# Autodesk Inventor assembly: Extrusions (1)
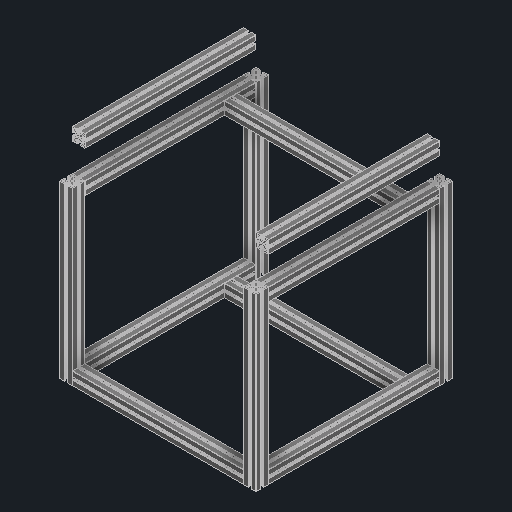
[picture p0: Inventor's stored thumbnail of the model, 512x512]
Saved by Autodesk Inventor 2025.1 (Build 291241020, 241B)
## iProperties
Created: 2025-05-09
Part Number: Extrusions (1)
Document SubType Name: Assembly
Designer: AdminForWorker
Title: Extrusions
Author: AdminForWorker
## Documents named in this file (7)
- C:\Users\Joshua Eah\Documents\Voron 0.2\CAD\Master Assembly\Extrusions (1).iam
- Extrusions.iam
- C:\Users\Joshua Eah\Documents\Voron 0.2\CAD\Master Assembly\Extrusions\1515_200mm - E.ipt
- C:\Users\Joshua Eah\Documents\Voron 0.2\CAD\Master Assembly\Extrusions\1515_200mm - C.ipt
- C:\Users\Joshua Eah\Documents\Voron 0.2\CAD\Master Assembly\Extrusions\1515_200mm - D.ipt
- C:\Users\Joshua Eah\Documents\Voron 0.2\CAD\Master Assembly\Extrusions\1515_200mm - B.ipt
- C:\Users\Joshua Eah\Documents\Voron 0.2\CAD\Master Assembly\Hardware\M3x8 BHCS.ipt
## Components (27 placed, 5 different names)
1. 1515_200mm - E:1 — Flush:1, Flush:2, Mate:13, Mate:48, Mate:51
2. 1515_200mm - C:1 — Mate:16, Mate:17, Mate:34, Mate:36, Flush:17
3. 1515_200mm - D:1 — Mate:7, Mate:8, Mate:29, Flush:7, Flush:8, Mate:30, Mate:35, Flush:14, Flush:15, Mate:37, Mate:38
4. 1515_200mm - B:1 — Mate:26, Mate:27, Flush:7, Flush:8, Mate:30, Mate:31, Flush:9, Flush:10
5. 1515_200mm - E:2 — Mate:20, Mate:21, Flush:14, Flush:15, Mate:38, Mate:41, Mate:45
6. 1515_200mm - D:2 — Mate:5, Mate:6, Flush:1, Flush:2, Mate:13, Mate:24, Mate:25, Flush:5, Flush:6, Mate:28, Mate:31, Flush:9, Flush:10
7. 1515_200mm - B:2
8. 1515_200mm - C:2 — Mate:14, Mate:15, Mate:22, Mate:23, Flush:3, Flush:4
9. 1515_200mm - B:3
10. 1515_200mm - B:4 — Mate:39, Mate:40, Mate:43, Flush:16
11. 1515_200mm - E:3 — Mate:32, Mate:33, Mate:34, Mate:35, Flush:17, Mate:49, Mate:50, Flush:18, Mate:52
12. 1515_200mm - B:5 — Mate:46, Mate:47, Flush:18, Mate:52
13. 1515_200mm - E:4 — Mate:18, Mate:19, Mate:23, Flush:3, Flush:4, Mate:25, Flush:5, Flush:6, Mate:42, Mate:43, Mate:44, Flush:16
14. M3x8 BHCS:1 — Mate:40, Mate:42, Mate:44
15. M3x8 BHCS:2 — Mate:27, Mate:28
16. M3x8 BHCS:3 — Mate:19, Mate:24
17. M3x8 BHCS:4 — Mate:20, Mate:37
18. M3x8 BHCS:5 — Mate:26, Mate:29
19. M3x8 BHCS:6 — Mate:39, Mate:41, Mate:45
20. M3x8 BHCS:7 — Mate:18, Mate:22
21. M3x8 BHCS:8 — Mate:21, Mate:36
22. M3x8 BHCS:9 — Mate:16, Mate:17, Mate:33
23. M3x8 BHCS:10 — Mate:5, Mate:6
24. M3x8 BHCS:11 — Mate:14, Mate:15
25. M3x8 BHCS:12 — Mate:7, Mate:8, Mate:32
26. M3x8 BHCS:13 — Mate:46, Mate:49, Mate:50
27. M3x8 BHCS:14 — Mate:47, Mate:48, Mate:51
## Relationships (59: Mate 44, Flush 15)
- Mate:5: 1515_200mm - D:2 ↔ M3x8 BHCS:10
- Mate:6: 1515_200mm - D:2 ↔ M3x8 BHCS:10
- Mate:7: 1515_200mm - D:1 ↔ M3x8 BHCS:12
- Mate:8: 1515_200mm - D:1 ↔ M3x8 BHCS:12
- Flush:1: 1515_200mm - E:1 ↔ 1515_200mm - D:2
- Flush:2: 1515_200mm - E:1 ↔ 1515_200mm - D:2
- Mate:13: 1515_200mm - E:1 ↔ 1515_200mm - D:2
- Mate:14: 1515_200mm - C:2 ↔ M3x8 BHCS:11
- Mate:15: 1515_200mm - C:2 ↔ M3x8 BHCS:11
- Mate:16: 1515_200mm - C:1 ↔ M3x8 BHCS:9
- Mate:17: 1515_200mm - C:1 ↔ M3x8 BHCS:9
- Mate:18: 1515_200mm - E:4 ↔ M3x8 BHCS:7
- Mate:19: 1515_200mm - E:4 ↔ M3x8 BHCS:3
- Mate:20: 1515_200mm - E:2 ↔ M3x8 BHCS:4
- Mate:21: 1515_200mm - E:2 ↔ M3x8 BHCS:8
- Mate:22: 1515_200mm - C:2 ↔ M3x8 BHCS:7
- Mate:23: 1515_200mm - C:2 ↔ 1515_200mm - E:4
- Flush:3: 1515_200mm - C:2 ↔ 1515_200mm - E:4
- Flush:4: 1515_200mm - C:2 ↔ 1515_200mm - E:4
- Mate:24: 1515_200mm - D:2 ↔ M3x8 BHCS:3
- Mate:25: 1515_200mm - D:2 ↔ 1515_200mm - E:4
- Flush:5: 1515_200mm - D:2 ↔ 1515_200mm - E:4
- Flush:6: 1515_200mm - D:2 ↔ 1515_200mm - E:4
- Mate:26: 1515_200mm - B:1 ↔ M3x8 BHCS:5
- Mate:27: 1515_200mm - B:1 ↔ M3x8 BHCS:2
- Mate:28: 1515_200mm - D:2 ↔ M3x8 BHCS:2
- Mate:29: 1515_200mm - D:1 ↔ M3x8 BHCS:5
- Flush:7: 1515_200mm - D:1 ↔ 1515_200mm - B:1
- Flush:8: 1515_200mm - D:1 ↔ 1515_200mm - B:1
- Mate:30: 1515_200mm - D:1 ↔ 1515_200mm - B:1
- Mate:31: 1515_200mm - B:1 ↔ 1515_200mm - D:2
- Flush:9: 1515_200mm - B:1 ↔ 1515_200mm - D:2
- Flush:10: 1515_200mm - B:1 ↔ 1515_200mm - D:2
- Mate:32: 1515_200mm - E:3 ↔ M3x8 BHCS:12
- Mate:33: 1515_200mm - E:3 ↔ M3x8 BHCS:9
- Mate:34: 1515_200mm - C:1 ↔ 1515_200mm - E:3
- Mate:35: 1515_200mm - D:1 ↔ 1515_200mm - E:3
- Flush:14: 1515_200mm - D:1 ↔ 1515_200mm - E:2
- Flush:15: 1515_200mm - D:1 ↔ 1515_200mm - E:2
- Mate:36: 1515_200mm - C:1 ↔ M3x8 BHCS:8
- Mate:37: 1515_200mm - D:1 ↔ M3x8 BHCS:4
- Mate:38: 1515_200mm - D:1 ↔ 1515_200mm - E:2
- Mate:39: 1515_200mm - B:4 ↔ M3x8 BHCS:6
- Mate:40: 1515_200mm - B:4 ↔ M3x8 BHCS:1
- Mate:41: 1515_200mm - E:2 ↔ M3x8 BHCS:6
- Mate:42: 1515_200mm - E:4 ↔ M3x8 BHCS:1
- Mate:43: 1515_200mm - B:4 ↔ 1515_200mm - E:4
- Mate:44: 1515_200mm - E:4 ↔ M3x8 BHCS:1
- Mate:45: 1515_200mm - E:2 ↔ M3x8 BHCS:6
- Flush:16: 1515_200mm - B:4 ↔ 1515_200mm - E:4
- Mate:46: 1515_200mm - B:5 ↔ M3x8 BHCS:13
- Mate:47: 1515_200mm - B:5 ↔ M3x8 BHCS:14
- Mate:48: 1515_200mm - E:1 ↔ M3x8 BHCS:14
- Flush:17: 1515_200mm - C:1 ↔ 1515_200mm - E:3
- Mate:49: 1515_200mm - E:3 ↔ M3x8 BHCS:13
- Mate:50: 1515_200mm - E:3 ↔ M3x8 BHCS:13
- Mate:51: 1515_200mm - E:1 ↔ M3x8 BHCS:14
- Flush:18: 1515_200mm - E:3 ↔ 1515_200mm - B:5
- Mate:52: 1515_200mm - E:3 ↔ 1515_200mm - B:5
